# Autodesk Inventor assembly: field
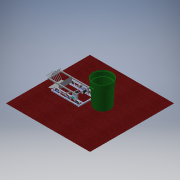
[picture p0: Inventor's stored thumbnail of the model, 180x180]
Saved by Autodesk Inventor 2016 (Build 200138000, 138)
## iProperties
Created: 2016-09-04
Part Number: field
Document SubType Name: Assembly
Designer: gus
Author: gus
## Documents named in this file (4)
- \\Mac\Home\Desktop\bunnybots 2016\prototype\field.iam
- \\Mac\Home\Desktop\bunnybots 2016\prototype\Assembly1.iam
- \\Mac\Home\Desktop\bunnybots 2016\prototype\Part8.ipt
- \\Mac\Home\Desktop\bunnybots 2016\prototype\RECYCLING_CAN.ipt
## Components (3 placed, 3 different names)
1. Assembly1:1 [sub-assembly] — Mate:2
2. Part8:1 — Mate:1, Mate:2
3. RECYCLING_CAN:1 — Mate:1
## Relationships (2: Mate 2)
- Mate:1: Part8:1 ↔ RECYCLING_CAN:1
- Mate:2 (63.5 mm): Assembly1:1 ↔ Part8:1
